# Autodesk Inventor assembly: ArmSquare
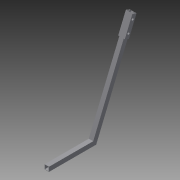
[picture p0: Inventor's stored thumbnail of the model, 180x180]
Saved by Autodesk Inventor 2013 (Build 170138000, 138)
## iProperties
Created: 2014-01-20
Part Number: ArmSquare
Document SubType Name: Assembly
Designer: RobertB
Author: RobertB
## Documents named in this file (4)
- E:\Robotics\FRC\2014\CAD\Robot\Catapult\ArmSquare.iam
- E:\Robotics\FRC\2014\CAD\Robot\Catapult\CatapultArmSquare-Bottom.ipt
- E:\Robotics\FRC\2014\CAD\Robot\Catapult\CatapultArmSquare-Top.ipt
- E:\Robotics\FRC\2014\CAD\Robot\Catapult\CatapultArmSquare-Thickener.ipt
## Components (4 placed, 3 different names)
1. CatapultArmSquare-Bottom:1 — Mate:1, Flush:1, Mate:2
2. CatapultArmSquare-Top:1 — Mate:1, Flush:1, Mate:2, Mate:3, Flush:2, Flush:3, Mate:4, Flush:5
3. CatapultArmSquare-Thickener:1 — Mate:4, Flush:4, Flush:5
4. CatapultArmSquare-Thickener:2 — Mate:3, Flush:2, Flush:3, Flush:4
## Relationships (9: Flush 5, Mate 4)
- Mate:1: CatapultArmSquare-Bottom:1 ↔ CatapultArmSquare-Top:1
- Flush:1: CatapultArmSquare-Bottom:1 ↔ CatapultArmSquare-Top:1
- Mate:2: CatapultArmSquare-Bottom:1 ↔ CatapultArmSquare-Top:1
- Mate:3: CatapultArmSquare-Top:1 ↔ CatapultArmSquare-Thickener:2
- Flush:2: CatapultArmSquare-Top:1 ↔ CatapultArmSquare-Thickener:2
- Flush:3: CatapultArmSquare-Top:1 ↔ CatapultArmSquare-Thickener:2
- Mate:4: CatapultArmSquare-Top:1 ↔ CatapultArmSquare-Thickener:1
- Flush:4: CatapultArmSquare-Thickener:1 ↔ CatapultArmSquare-Thickener:2
- Flush:5: CatapultArmSquare-Top:1 ↔ CatapultArmSquare-Thickener:1
